# Autodesk Inventor assembly: S5
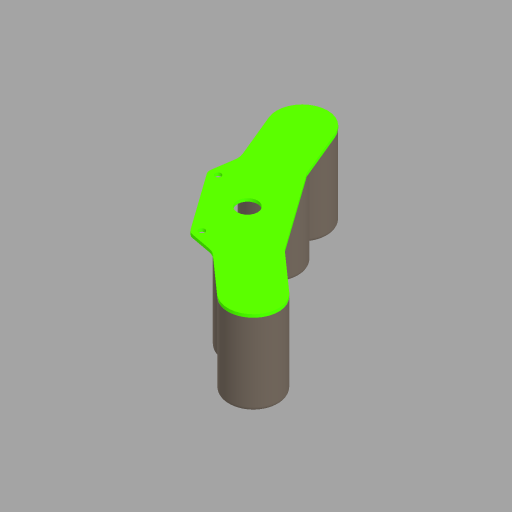
[picture p0: Inventor's stored thumbnail of the model, 512x512]
Saved by Autodesk Inventor 2024.2 (Build 282272000, 272)
## iProperties
Created: 2024-01-20
Part Number: S5
Document SubType Name: Assembly
Designer: Fedor Orlov
Author: Fedor Orlov
## Documents named in this file (3)
- C:\Users\Fedor Orlov\OneDrive\Robocup SSL\3D model\S5.iam
- C:\Users\Fedor Orlov\OneDrive\Robocup SSL\3D model\Capasitor_board.ipt
- C:\Users\Fedor Orlov\OneDrive\Robocup SSL\3D model\Capasitor.ipt
## Components (5 placed, 2 different names)
1. Capasitor_board:1 — Совмещение:1, Совмещение:2, Совмещение:3, Касательность:1, Совмещение:5, Совмещение:6, Совмещение:7, Касательность:2
2. Capasitor:1 — Совмещение:1, Совмещение:2, Совмещение:4
3. Capasitor:2 — Совмещение:3, Касательность:1, Совмещение:4
4. Capasitor:3 — Совмещение:5, Совмещение:7, Совмещение:8
5. Capasitor:4 — Совмещение:6, Касательность:2, Совмещение:8
## Relationships (10: Mate 8, Tangent 2)
- Совмещение:1 [Mate]: Capasitor_board:1 ↔ Capasitor:1
- Совмещение:2 [Mate]: Capasitor_board:1 ↔ Capasitor:1
- Совмещение:3 [Mate]: Capasitor_board:1 ↔ Capasitor:2
- Касательность:1 [Tangent]: Capasitor_board:1 ↔ Capasitor:2
- Совмещение:4 [Mate] (26 mm): Capasitor:1 ↔ Capasitor:2
- Совмещение:5 [Mate]: Capasitor_board:1 ↔ Capasitor:3
- Совмещение:6 [Mate]: Capasitor_board:1 ↔ Capasitor:4
- Совмещение:7 [Mate]: Capasitor_board:1 ↔ Capasitor:3
- Касательность:2 [Tangent]: Capasitor_board:1 ↔ Capasitor:4
- Совмещение:8 [Mate] (26 mm): Capasitor:3 ↔ Capasitor:4
